# Autodesk Inventor assembly: Piston_Rod
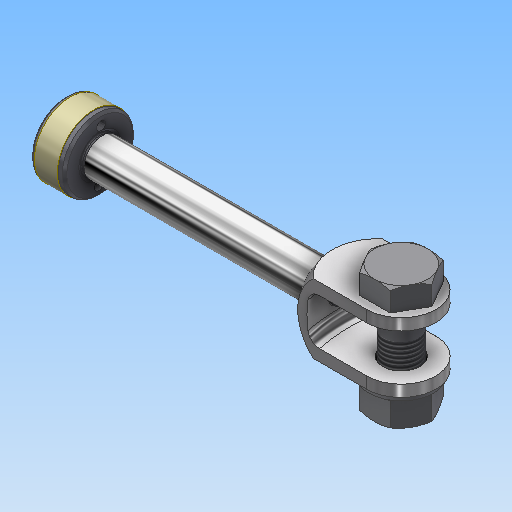
[picture p0: Inventor's stored thumbnail of the model, 512x512]
Saved by Autodesk Inventor 2020.1 (Build 241239000, 239)
## iProperties
Created: 2003-05-03
Part Number: Piston_Rod
Document SubType Name: Assembly
Designer: Stephen Hooper
Manufacturer: Standard
Standards Organization: Custom
Control State: 0
Master: False
Checked Out: False
Shininess: 64.0
Length Units: 11269
Angle Units: 11279
Time Units: 11290
Mass Units: 11283
Length Display Precision: 3
Angle Display Precision: 2
Compacted: True
Density: 0.0
Volumn: 0.0
Area: 0.0
PropertySet Name: Model Information
Author: Stephen Hooper
## Documents named in this file (8)
- C:\Users\thomastremblay\Desktop\Inventor ACP Data\Assemblies\Piston_Rod.iam
- C:\Users\thomastremblay\Desktop\Inventor ACP Data\Parts\Piston_Rod.ipt
- C:\Users\thomastremblay\Desktop\Inventor ACP Data\Parts\Piston_Plunger.ipt
- C:\Users\thomastremblay\Desktop\Inventor ACP Data\Parts\Plunger_Seal.ipt
- C:\Users\thomastremblay\Desktop\Inventor ACP Data\Parts\Piston_Connector.ipt
- C:\Users\thomastremblay\Desktop\Inventor ACP Data\Content Center\local.BSI.47.140.5.ipt
- C:\Users\thomastremblay\Desktop\Inventor ACP Data\Content Center\local.BSI.30.190.5.ipt
- C:\Users\thomastremblay\Desktop\Inventor ACP Data\Content Center\local.BSI.6.3030.5.ipt
## Components (7 placed, 7 different names)
1. Piston_Rod:1 — Mate:3, Mate:4, Mate:5, Mate:6
2. Piston_Plunger:1 — Mate:1, Mate:2, Mate:3, Mate:6
3. Plunger_Seal:1 — Mate:1, Mate:2
4. Piston_Connector:2 — Mate:4, Mate:5, Insert:1, Insert:2
5. BS 3692  Hexagon Head Screw  (Regular Thread - Metric) M30 x 90:1 — Insert:1
6. BS 4320  Form E M30 (Form E):1 — Insert:2, Insert:3
7. BS 3692  (Regular Thread - Metric) M30:1 — Insert:3
## Relationships (9: Mate 6, Insert 3)
- Mate:1: Piston_Plunger:1 ↔ Plunger_Seal:1
- Mate:2: Piston_Plunger:1 ↔ Plunger_Seal:1
- Mate:3: Piston_Rod:1 ↔ Piston_Plunger:1
- Mate:4: Piston_Rod:1 ↔ Piston_Connector:2
- Mate:5: Piston_Rod:1 ↔ Piston_Connector:2
- Insert:1: Piston_Connector:2 ↔ BS 3692  Hexagon Head Screw  (Regular Thread - Metric) M30 x 90:1
- Insert:2: Piston_Connector:2 ↔ BS 4320  Form E M30 (Form E):1
- Insert:3: BS 4320  Form E M30 (Form E):1 ↔ BS 3692  (Regular Thread - Metric) M30:1
- Mate:6: Piston_Rod:1 ↔ Piston_Plunger:1
